# Autodesk Inventor assembly: Trunk
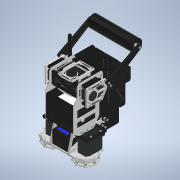
[picture p0: Inventor's stored thumbnail of the model, 180x180]
Saved by Autodesk Inventor 2020.4 (Build 244396000, 396)
## iProperties
Created: 2021-09-10
Part Number: Trunk
Document SubType Name: Assembly
Designer: Masato
Mass: 1705.67 g
Surface Area: 5977.9 cm^2
Volume: 961.439 cm^3
Density: 1.77408 g/cm^3
Author: Masato
## Documents named in this file (38)
- C:\Users\Masato\Documents\Inventor\CIT Brains_Inventor\OpenPlatform_ver3_0\UpperBody\Trunk\Trunk.iam
- C:\Users\Masato\Documents\Inventor\CIT Brains_Inventor\OpenPlatform_ver3_0\UpperBody\Trunk\Trunk_horizontal_frame_03.ipt
- C:\Users\Masato\Documents\Inventor\CIT Brains_Inventor\OpenPlatform_ver3_0\UpperBody\Trunk\Trunk_horizontal_frame_04.ipt
- C:\Users\Masato\Documents\Inventor\CIT Brains_Inventor\OpenPlatform_ver3_0\UpperBody\Trunk\Trunk_horizontal_frame_05.ipt
- C:\Users\Masato\Documents\Inventor\CIT Brains_Inventor\OpenPlatform_ver3_0\UpperBody\Trunk\Trunk_vertical_frame_02.ipt
- C:\Users\Masato\Documents\Inventor\CIT Brains_Inventor\OpenPlatform_ver3_0\UpperBody\Trunk\Trunk_vertical_frame_03.ipt
- C:\Users\Masato\Documents\Inventor\CIT Brains_Inventor\OpenPlatform_ver3_0\UpperBody\Trunk\Trunk_vertical_frame_04.ipt
- C:\Users\Masato\Documents\Inventor\CIT Brains_Inventor\OpenPlatform_ver3_0\UpperBody\Trunk\Trunk_vertical_frame_05.ipt
- C:\Users\Masato\Documents\Inventor\CIT Brains_Inventor\OpenPlatform_ver3_0\UpperBody\Trunk\Trunk_vertical_frame_06.ipt
- C:\Users\Masato\Documents\Inventor\CIT Brains_Inventor\OpenPlatform_ver3_0\Ready_Made\B3M11xx.ipt
- C:\Users\Masato\Documents\Inventor\CIT Brains_Inventor\OpenPlatform_ver3_0\Ready_Made\S3-07-3W.ipt
- C:\Users\Masato\Documents\Inventor\CIT Brains_Inventor\OpenPlatform_ver3_0\Ready_Made\ASU-375H.ipt
- C:\Users\Masato\Documents\Inventor\CIT Brains_Inventor\OpenPlatform_ver3_0\Ready_Made\B3M10xx.ipt
- C:\Users\Masato\Documents\Inventor\CIT Brains_Inventor\OpenPlatform_ver3_0\Ready_Made\SGB-100.ipt
- C:\Users\Masato\Documents\Inventor\CIT Brains_Inventor\OpenPlatform_ver3_0\UpperBody\Cockpit\Cockpit.iam
- C:\Users\Masato\Documents\Inventor\CIT Brains_Inventor\OpenPlatform_ver3_0\UpperBody\Trunk\Trunk_vertical_frame_04_MIR.ipt
- C:\Users\Masato\Documents\Inventor\CIT Brains_Inventor\OpenPlatform_ver3_0\UpperBody\Trunk\Trunk_vertical_frame_01.ipt
- C:\Users\Masato\Documents\Inventor\CIT Brains_Inventor\OpenPlatform_ver3_0\UpperBody\Trunk\Trunk_vertical_frame_01_MIR.ipt
- C:\Users\Masato\Documents\Inventor\CIT Brains_Inventor\OpenPlatform_ver3_0\Ready_Made\Screw\SPNFL-BRN-M3-6.ipt
- C:\Users\Masato\Documents\Inventor\CIT Brains_Inventor\OpenPlatform_ver3_0\Ready_Made\Screw\M2_6-15.ipt
- C:\Users\Masato\Documents\Inventor\CIT Brains_Inventor\OpenPlatform_ver3_0\Ready_Made\Screw\M3-8.ipt
- C:\Users\Masato\Documents\Inventor\CIT Brains_Inventor\OpenPlatform_ver3_0\Ready_Made\Screw\M3-6.ipt
- C:\Users\Masato\Documents\Inventor\CIT Brains_Inventor\OpenPlatform_ver3_0\Ready_Made\Screw\M2_6-20.ipt
- C:\Users\Masato\Documents\Inventor\CIT Brains_Inventor\OpenPlatform_ver3_0\UpperBody\Trunk\Outer_support_stand.ipt
- C:\Users\Masato\Documents\Inventor\CIT Brains_Inventor\OpenPlatform_ver3_0\Ready_Made\BRU-307S.ipt
- C:\Users\Masato\Documents\Inventor\CIT Brains_Inventor\OpenPlatform_ver3_0\UpperBody\Trunk\Outer_flange.ipt
- C:\Users\Masato\Documents\Inventor\CIT Brains_Inventor\OpenPlatform_ver3_0\UpperBody\Trunk\Inner_flange.ipt
- C:\Users\Masato\Documents\Inventor\CIT Brains_Inventor\OpenPlatform_ver3_0\Ready_Made\CRBA02508WWC8P5\CRBA02508WWC8P5.ipt
- C:\Users\Masato\Documents\Inventor\CIT Brains_Inventor\OpenPlatform_ver3_0\UpperBody\Trunk\Inner_support_stand.ipt
- C:\Users\Masato\Documents\Inventor\CIT Brains_Inventor\OpenPlatform_ver3_0\UpperBody\Trunk\Trunk_horizontal_frame_01.ipt
- C:\Users\Masato\Documents\Inventor\CIT Brains_Inventor\OpenPlatform_ver3_0\Ready_Made\SF319.ipt
- C:\Users\Masato\Documents\Inventor\CIT Brains_Inventor\OpenPlatform_ver3_0\Ready_Made\BRU-2609S.ipt
- C:\Users\Masato\Documents\Inventor\CIT Brains_Inventor\OpenPlatform_ver3_0\Ready_Made\Screw\M2_6-8.ipt
- C:\Users\Masato\Documents\Inventor\CIT Brains_Inventor\OpenPlatform_ver3_0\UpperBody\Trunk\Trunk_horizontal_frame_02.ipt
- C:\Users\Masato\Documents\Inventor\CIT Brains_Inventor\OpenPlatform_ver3_0\Ready_Made\UUW-0312-10BH.ipt
- C:\Users\Masato\Documents\Inventor\CIT Brains_Inventor\OpenPlatform_ver3_0\Ready_Made\Screw\M2_6-6.ipt
- C:\Users\Masato\Documents\Inventor\CIT Brains_Inventor\OpenPlatform_ver3_0\Ready_Made\ASU-309-6.ipt
- C:\Users\Masato\Documents\Inventor\CIT Brains_Inventor\OpenPlatform_ver3_0\Ready_Made\SLSBF7-131-M3-N3.ipt
## Components (229 placed, 37 different names)
1. Trunk_horizontal_frame_03:1 — 挿入:172, 挿入:173, 挿入:174, 挿入:175, 挿入:177, 挿入:179, 挿入:255, 挿入:256, 挿入:261, 挿入:262, 挿入:347, 挿入:348, 挿入:463, 挿入:464
2. Trunk_horizontal_frame_03:2 — 挿入:181, 挿入:182, 挿入:184, 挿入:185, 挿入:186, 挿入:187, 挿入:257, 挿入:258, 挿入:337, 挿入:338, 挿入:465, 挿入:466
3. Trunk_horizontal_frame_04:1 — 挿入:115, 挿入:116, 挿入:117, 挿入:118, 挿入:172, 挿入:173, 挿入:181, 挿入:182
4. Trunk_horizontal_frame_04:2 — 挿入:154, 挿入:155, 挿入:156, 挿入:157, 挿入:174, 挿入:175, 挿入:185, 挿入:187
5. Trunk_horizontal_frame_05:1 — 挿入:111, 挿入:112, 挿入:555, 挿入:556
6. Trunk_horizontal_frame_05:2 — 挿入:164, 挿入:165, 挿入:557, 挿入:558
7. Trunk_horizontal_frame_05:3 — 挿入:229, 挿入:230, 挿入:577, 挿入:579
8. Trunk_horizontal_frame_05:4 — 挿入:168, 挿入:169, 挿入:578, 挿入:580
9. Trunk_vertical_frame_01:1 — 角度:35, 角度:36, 挿入:200, 挿入:201, 挿入:420, 挿入:421, 挿入:426, 挿入:501, 挿入:502
10. Trunk_vertical_frame_01_MIR:1 — 角度:37, 角度:38, 挿入:202, 挿入:203, メイト:23, メイト:24, メイト:25, 挿入:418, 挿入:419, 挿入:499, 挿入:500
11. Trunk_vertical_frame_02:1 — フラッシュ:16, メイト:17, フラッシュ:18, フラッシュ:20, フラッシュ:21, メイト:22
12. Trunk_vertical_frame_02:2 — フラッシュ:16, メイト:17, フラッシュ:18, メイト:19
13. Trunk_vertical_frame_02:3 — フラッシュ:15, メイト:18, フラッシュ:17, フラッシュ:19, フラッシュ:20, フラッシュ:21, メイト:21, メイト:20
14. Trunk_vertical_frame_02:4 — フラッシュ:15, メイト:18, フラッシュ:17, メイト:25
15. Trunk_vertical_frame_03:1 — 挿入:101, 挿入:102, 挿入:103, 挿入:111, 挿入:112, 挿入:115, 挿入:116, 挿入:156, 挿入:157, 挿入:164, 挿入:165, フラッシュ:19, メイト:21, 挿入:208, 挿入:226, 挿入:245, 挿入:246, 挿入:247, 挿入:251, 挿入:252, 挿入:327, 挿入:328, 挿入:329, 挿入:330, 挿入:349, 挿入:350
16. Trunk_vertical_frame_03:2 — 挿入:104, 挿入:105, 挿入:106, 挿入:117, 挿入:118, 挿入:154, 挿入:155, 挿入:168, 挿入:169, メイト:22, 挿入:227, 挿入:229, 挿入:230, 挿入:248, 挿入:249, 挿入:250, 挿入:253, 挿入:254, 挿入:331, 挿入:332, 挿入:333, 挿入:334, 挿入:351, 挿入:352
17. Trunk_vertical_frame_04:1 — 挿入:555, 挿入:556, 挿入:557, 挿入:558, 挿入:559, 挿入:560, 挿入:561, 挿入:562, 挿入:563, 挿入:564, 挿入:565, 挿入:566, 挿入:567, 挿入:568, 挿入:569, 挿入:570, 角度:48, 挿入:571, 角度:49, 挿入:572, 挿入:573, 挿入:574
18. Trunk_vertical_frame_04_MIR:1 — 挿入:577, 挿入:578, 挿入:579, 挿入:580, 挿入:581, 挿入:582, 挿入:583, 挿入:584, 挿入:585, 挿入:586, 挿入:587, 挿入:588, 挿入:589, 挿入:590, 挿入:591, 挿入:592, 挿入:593, 挿入:594, 角度:50, 角度:51, 挿入:595, 挿入:596
19. Trunk_vertical_frame_05:1 — メイト:16, 挿入:263, 挿入:264, 挿入:267, 挿入:575, 挿入:576, 角度:52, 挿入:599
20. Trunk_vertical_frame_05:2 — 挿入:265, 挿入:266, 挿入:268, 挿入:597, 挿入:598
21. Trunk_vertical_frame_06:1 — 挿入:467, 挿入:468, 挿入:469, 挿入:470, 挿入:471, 挿入:472, 挿入:473, 挿入:474
22. Trunk_vertical_frame_06:2 — 挿入:475, 挿入:476, 挿入:477, 挿入:478, 挿入:479, 挿入:480, 挿入:481, 挿入:482
23. B3M11xx:1 — 角度:39, 挿入:391, 挿入:392, 挿入:422, 挿入:423, 挿入:424, 挿入:425, 挿入:483, 挿入:486
24. B3M11xx:2 — 挿入:427, 挿入:428, 挿入:429, 挿入:484, 挿入:485, 挿入:529
25. B3M11xx:3 — 挿入:177, 挿入:179, 挿入:184, 挿入:186
26. B3M10xx:4 — 挿入:475, 挿入:476, 挿入:477, 挿入:478, 挿入:559, 挿入:560, 挿入:561, 挿入:562
27. B3M10xx:5 — 挿入:467, 挿入:468, 挿入:469, 挿入:470, 挿入:581, 挿入:582, 挿入:583, 挿入:584
28. S3-07-3W:1 — 角度:37, 挿入:202
29. S3-07-3W:2 — 角度:38, 挿入:203
30. S3-07-3W:3 — 角度:36, 挿入:201
31. S3-07-3W:4 — 角度:35, 挿入:200
32. ASU-375H:1 — フラッシュ:9, フラッシュ:10, フラッシュ:11, フラッシュ:12, 挿入:101, 挿入:104, メイト:19, メイト:20, メイト:23, メイト:24
33. ASU-375H:2 — フラッシュ:9, フラッシュ:11, 挿入:102, 挿入:105
34. ASU-375H:3 — フラッシュ:10, フラッシュ:12, 挿入:103, 挿入:106
35. SGB-100:1 — メイト:16
36. Cockpit:1 [sub-assembly] — 挿入:208, 角度:39
37. SPNFL-BRN-M3-6:1 — 挿入:226
38. SPNFL-BRN-M3-6:2 — 挿入:227
39. M3-8:5 — 挿入:245
40. M3-8:6 — 挿入:246
41. M3-8:7 — 挿入:247
42. M3-8:8 — 挿入:248
43. M3-8:9 — 挿入:249
44. M3-8:10 — 挿入:250
45. M3-6:1 — 挿入:251
46. M3-6:2 — 挿入:252
47. M3-6:3 — 挿入:254
48. M3-6:4 — 挿入:253
49. M3-6:5 — 挿入:256
50. M3-6:6 — 挿入:255
51. M3-6:7 — 挿入:258
52. M3-6:8 — 挿入:257
53. M2_6-15:9 — 挿入:464
54. M2_6-15:10 — 挿入:463
55. M2_6-15:11 — 挿入:261
56. M2_6-15:12 — 挿入:262
57. M3-6:9 — 挿入:263
58. M3-6:10 — 挿入:264
59. M3-6:11 — 挿入:266
60. M3-6:12 — 挿入:265
61. M3-8:11 — 挿入:267
62. M3-8:12 — 挿入:268
63. M2_6-20:1 — 挿入:489
64. M2_6-20:2 — 挿入:490
65. M2_6-20:3 — 挿入:487
66. M2_6-20:4 — 挿入:488
67. M2_6-15:13 — 挿入:564
68. M2_6-15:14 — 挿入:563
69. M2_6-15:15 — 挿入:566
70. M2_6-15:16 — 挿入:565
71. M2_6-15:17 — 挿入:591
72. M2_6-15:18 — 挿入:592
73. M2_6-15:19 — 挿入:589
74. M2_6-15:20 — 挿入:590
75. M3-6:13 — 挿入:567
76. M3-6:14 — 挿入:568
77. M3-6:15 — 挿入:569
78. M3-6:16 — 挿入:570
79. M3-6:17 — 挿入:585
80. M3-6:18 — 挿入:586
81. M3-6:19 — 挿入:587
82. M3-6:20 — 挿入:588
83. M3-6:21 — 挿入:327
84. M3-6:22 — 挿入:328
85. M3-6:23 — 挿入:329
86. M3-6:24 — 挿入:330
87. M3-6:25 — 挿入:331
88. M3-6:26 — 挿入:332
89. M3-6:27 — 挿入:333
90. M3-6:28 — 挿入:334
91. M2_6-20:9 — 挿入:465
92. M2_6-20:10 — 挿入:466
93. M2_6-20:11 — 挿入:337
94. M2_6-20:12 — 挿入:338
95. M2_6-20:13 — 挿入:479
96. M2_6-20:14 — 挿入:482
97. M2_6-20:15 — 挿入:481
98. M2_6-20:16 — 挿入:480
99. M2_6-20:17 — 挿入:474
100. M2_6-20:18 — 挿入:472
101. M2_6-20:19 — 挿入:473
102. M2_6-20:20 — 挿入:471
103. M3-6:29 — 挿入:347
104. M3-6:30 — 挿入:348
105. M3-6:31 — 挿入:349
106. M3-6:32 — 挿入:350
107. M3-6:33 — 挿入:351
108. M3-6:34 — 挿入:352
109. Outer_support_stand:1 — 挿入:371, 挿入:372, 挿入:373, 挿入:374, 挿入:375, 挿入:376, 挿入:377, 挿入:378, 挿入:397, 挿入:438, 挿入:439
110. BRU-307S:1 — 挿入:371, 挿入:404
111. BRU-307S:2 — 挿入:372
112. BRU-307S:3 — 挿入:373
113. BRU-307S:4 — 挿入:374
114. BRU-307S:5 — 挿入:375, 挿入:405
115. BRU-307S:6 — 挿入:376
116. BRU-307S:7 — 挿入:377
117. BRU-307S:8 — 挿入:378
118. Inner_flange:1 — 挿入:391, 挿入:392, 挿入:452, 挿入:453, 挿入:454, 挿入:455
119. CRBA02508WWC8P5:1 — 挿入:397
120. Inner_support_stand:1 — 角度:40, 挿入:398, 角度:41, 挿入:399, 角度:42, 挿入:400, 角度:43, 挿入:401, 挿入:456, 挿入:457, 挿入:458, 挿入:459, 挿入:460, 挿入:461
121. S3-07-3W:9 — 角度:40, 挿入:398
122. S3-07-3W:10 — 角度:41, 挿入:399
123. S3-07-3W:11 — 角度:42, 挿入:400
124. S3-07-3W:12 — 角度:43, 挿入:401
125. Outer_flange:1 — 挿入:404, 挿入:405, 挿入:406, 挿入:407, 挿入:408, 挿入:409, 挿入:410, 挿入:411, 挿入:412, 挿入:413
126. M3-6:35 — 挿入:406
127. M3-6:36 — 挿入:407
128. M3-6:37 — 挿入:408
129. M3-6:38 — 挿入:409
130. M3-6:39 — 挿入:410
131. M3-6:40 — 挿入:411
132. M3-6:41 — 挿入:412
133. M3-6:42 — 挿入:413
134. Trunk_horizontal_frame_01:1 — 挿入:418, 挿入:419, 挿入:420, 挿入:421, 挿入:422, 挿入:423, 挿入:424, 挿入:425, 挿入:426, 挿入:427, 挿入:428, 挿入:429, 挿入:430, 挿入:431, 挿入:432, 挿入:433, 挿入:434, 挿入:435, 挿入:436, 挿入:440, 挿入:441, 挿入:442, 挿入:443, 挿入:444, 挿入:445, 挿入:446, 挿入:447, 挿入:448, 挿入:449, 挿入:450, 挿入:451, フラッシュ:22, 挿入:462, 挿入:511, 挿入:512, 挿入:513, 挿入:514, 挿入:515, 挿入:516, 挿入:517, 挿入:518
135. SF319:1 — 挿入:430
136. SF319:2 — 挿入:431
137. SF319:3 — 挿入:432
138. SF319:4 — 挿入:433, 挿入:439
139. SF319:5 — 挿入:434
140. SF319:6 — 挿入:435
141. SF319:7 — 挿入:436, 挿入:438
142. SF319:8 — 挿入:462
143. M2_6-15:21 — 挿入:441
144. M2_6-15:22 — 挿入:440
145. M2_6-15:23 — 挿入:442
146. M2_6-15:24 — 挿入:443
147. M2_6-15:25 — 挿入:444
148. M2_6-15:26 — 挿入:445
149. M2_6-15:27 — 挿入:446
150. M2_6-15:28 — 挿入:447
151. M3-8:13 — 挿入:448
152. M3-8:14 — 挿入:449
153. M3-8:15 — 挿入:450
154. M3-8:16 — 挿入:451
155. BRU-2609S:1 — 挿入:455, 挿入:457
156. BRU-2609S:2 — 挿入:454
157. BRU-2609S:3 — 挿入:453
158. BRU-2609S:4 — 挿入:452, 挿入:456
159. M2_6-8:1 — 挿入:458
160. M2_6-8:2 — 挿入:459
161. M2_6-8:3 — 挿入:460
162. M2_6-8:4 — 挿入:461
163. Trunk_horizontal_frame_02:1 — 挿入:483, 挿入:484, 挿入:485, 挿入:486, 挿入:487, 挿入:488, 挿入:489, 挿入:490
164. BRU-307S:9 — 挿入:497, 挿入:503
165. BRU-307S:10 — 挿入:498, 挿入:504
166. BRU-307S:11 — 挿入:496, 挿入:506
167. BRU-307S:12 — 挿入:495, 挿入:505
168. UUW-0312-10BH:1 — 挿入:495, 挿入:507
169. UUW-0312-10BH:2 — 挿入:496, 挿入:508
170. UUW-0312-10BH:3 — 挿入:497, 挿入:509
171. UUW-0312-10BH:4 — 挿入:498, 挿入:510
172. UUW-0312-10BH:5 — 挿入:499, 挿入:505
173. UUW-0312-10BH:6 — 挿入:500, 挿入:506
174. UUW-0312-10BH:7 — 挿入:501, 挿入:503
175. UUW-0312-10BH:8 — 挿入:502, 挿入:504
176. M3-6:43 — 挿入:507
177. M3-6:44 — 挿入:508
178. M3-6:45 — 挿入:510
179. M3-6:46 — 挿入:509
180. SF319:9 — 挿入:511, 挿入:519
181. SF319:10 — 挿入:512
182. SF319:11 — 挿入:513
183. SF319:12 — 挿入:514
184. SF319:13 — 挿入:515, 挿入:520
185. SF319:14 — 挿入:516
186. SF319:15 — 挿入:517
187. SF319:16 — 挿入:518
188. Outer_support_stand:2 — 挿入:519, 挿入:520, 挿入:521, 挿入:522, 挿入:523, 挿入:524, 挿入:525, 挿入:526, 挿入:527, 挿入:528, 挿入:554
189. BRU-307S:13 — 挿入:521, 挿入:534
190. BRU-307S:14 — 挿入:522
191. BRU-307S:15 — 挿入:523
192. BRU-307S:16 — 挿入:524
193. BRU-307S:17 — 挿入:525, 挿入:535
194. BRU-307S:18 — 挿入:526
195. BRU-307S:19 — 挿入:527
196. BRU-307S:20 — 挿入:528
197. BRU-2609S:5 — 挿入:530, 挿入:540
198. BRU-2609S:6 — 挿入:531, 挿入:541
199. BRU-2609S:7 — 挿入:532
200. BRU-2609S:8 — 挿入:533
201. S3-07-3W:13 — 角度:44, 挿入:536
202. S3-07-3W:14 — 角度:45, 挿入:537
203. S3-07-3W:15 — 角度:46, 挿入:538
204. S3-07-3W:16 — 角度:47, 挿入:539
205. Inner_flange:2 — 挿入:529, 挿入:530, 挿入:531, 挿入:532, 挿入:533
206. Inner_support_stand:2 — 角度:44, 挿入:536, 角度:45, 挿入:537, 角度:46, 挿入:538, 角度:47, 挿入:539, 挿入:540, 挿入:541, 挿入:550, 挿入:551, 挿入:552, 挿入:553
207. Outer_flange:2 — 挿入:534, 挿入:535, 挿入:542, 挿入:543, 挿入:544, 挿入:545, 挿入:546, 挿入:547, 挿入:548, 挿入:549
208. M3-6:47 — 挿入:542
209. M3-6:48 — 挿入:543
210. M3-6:49 — 挿入:544
211. M3-6:50 — 挿入:545
212. M3-6:51 — 挿入:546
213. M3-6:52 — 挿入:547
214. M3-6:53 — 挿入:548
215. M3-6:54 — 挿入:549
216. M2_6-6:1 — 挿入:550
217. M2_6-6:2 — 挿入:551
218. M2_6-6:3 — 挿入:552
219. M2_6-6:4 — 挿入:553
220. CRBA02508WWC8P5:2 — 挿入:554
221. ASU-309-6:1 — 角度:48, 挿入:571, 挿入:576
222. ASU-309-6:2 — 角度:49, 挿入:572, 挿入:575
223. M3-6:55 — 挿入:573
224. M3-6:56 — 挿入:574
225. M3-6:57 — 挿入:593
226. M3-6:58 — 挿入:594
227. ASU-309-6:3 — 角度:50, 挿入:595, 挿入:597
228. ASU-309-6:4 — 角度:51, 挿入:596, 挿入:598
229. SLSBF7-131-M3-N3:1 — 角度:52, 挿入:599
## Relationships (321: Insert 281, Angle 18, Flush 12, Mate 10)
- フラッシュ:9 [Flush]: ASU-375H:1 ↔ ASU-375H:2
- フラッシュ:10 [Flush]: ASU-375H:1 ↔ ASU-375H:3
- フラッシュ:11 [Flush]: ASU-375H:1 ↔ ASU-375H:2
- フラッシュ:12 [Flush]: ASU-375H:1 ↔ ASU-375H:3
- メイト:16 [Mate] (4 mm): Trunk_vertical_frame_05:1 ↔ SGB-100:1
- 挿入:101 [Insert]: Trunk_vertical_frame_03:1 ↔ ASU-375H:1
- 挿入:102 [Insert]: Trunk_vertical_frame_03:1 ↔ ASU-375H:2
- 挿入:103 [Insert]: Trunk_vertical_frame_03:1 ↔ ASU-375H:3
- 挿入:104 [Insert]: Trunk_vertical_frame_03:2 ↔ ASU-375H:1
- 挿入:105 [Insert]: Trunk_vertical_frame_03:2 ↔ ASU-375H:2
- 挿入:106 [Insert]: Trunk_vertical_frame_03:2 ↔ ASU-375H:3
- 挿入:111 [Insert]: Trunk_horizontal_frame_05:1 ↔ Trunk_vertical_frame_03:1
- 挿入:112 [Insert]: Trunk_horizontal_frame_05:1 ↔ Trunk_vertical_frame_03:1
- 挿入:115 [Insert]: Trunk_horizontal_frame_04:1 ↔ Trunk_vertical_frame_03:1
- 挿入:116 [Insert]: Trunk_horizontal_frame_04:1 ↔ Trunk_vertical_frame_03:1
- 挿入:117 [Insert]: Trunk_horizontal_frame_04:1 ↔ Trunk_vertical_frame_03:2
- 挿入:118 [Insert]: Trunk_horizontal_frame_04:1 ↔ Trunk_vertical_frame_03:2
- 挿入:154 [Insert]: Trunk_horizontal_frame_04:2 ↔ Trunk_vertical_frame_03:2
- 挿入:155 [Insert]: Trunk_horizontal_frame_04:2 ↔ Trunk_vertical_frame_03:2
- 挿入:156 [Insert]: Trunk_horizontal_frame_04:2 ↔ Trunk_vertical_frame_03:1
- 挿入:157 [Insert]: Trunk_horizontal_frame_04:2 ↔ Trunk_vertical_frame_03:1
- 挿入:164 [Insert]: Trunk_horizontal_frame_05:2 ↔ Trunk_vertical_frame_03:1
- 挿入:165 [Insert]: Trunk_horizontal_frame_05:2 ↔ Trunk_vertical_frame_03:1
- 挿入:168 [Insert]: Trunk_horizontal_frame_05:4 ↔ Trunk_vertical_frame_03:2
- 挿入:169 [Insert]: Trunk_horizontal_frame_05:4 ↔ Trunk_vertical_frame_03:2
- 挿入:172 [Insert]: Trunk_horizontal_frame_03:1 ↔ Trunk_horizontal_frame_04:1
- 挿入:173 [Insert]: Trunk_horizontal_frame_03:1 ↔ Trunk_horizontal_frame_04:1
- 挿入:174 [Insert]: Trunk_horizontal_frame_03:1 ↔ Trunk_horizontal_frame_04:2
- 挿入:175 [Insert]: Trunk_horizontal_frame_03:1 ↔ Trunk_horizontal_frame_04:2
- 挿入:177 [Insert]: Trunk_horizontal_frame_03:1 ↔ B3M11xx:3
- 挿入:179 [Insert]: Trunk_horizontal_frame_03:1 ↔ B3M11xx:3
- 挿入:181 [Insert]: Trunk_horizontal_frame_03:2 ↔ Trunk_horizontal_frame_04:1
- 挿入:182 [Insert]: Trunk_horizontal_frame_03:2 ↔ Trunk_horizontal_frame_04:1
- 挿入:184 [Insert]: Trunk_horizontal_frame_03:2 ↔ B3M11xx:3
- 挿入:185 [Insert]: Trunk_horizontal_frame_03:2 ↔ Trunk_horizontal_frame_04:2
- 挿入:186 [Insert]: Trunk_horizontal_frame_03:2 ↔ B3M11xx:3
- 挿入:187 [Insert]: Trunk_horizontal_frame_03:2 ↔ Trunk_horizontal_frame_04:2
- フラッシュ:15 [Flush]: Trunk_vertical_frame_02:3 ↔ Trunk_vertical_frame_02:4
- フラッシュ:16 [Flush]: Trunk_vertical_frame_02:1 ↔ Trunk_vertical_frame_02:2
- メイト:17 [Mate]: Trunk_vertical_frame_02:1 ↔ Trunk_vertical_frame_02:2
- メイト:18 [Mate]: Trunk_vertical_frame_02:3 ↔ Trunk_vertical_frame_02:4
- フラッシュ:17 [Flush]: Trunk_vertical_frame_02:3 ↔ Trunk_vertical_frame_02:4
- フラッシュ:18 [Flush]: Trunk_vertical_frame_02:1 ↔ Trunk_vertical_frame_02:2
- フラッシュ:19 [Flush]: Trunk_vertical_frame_02:3 ↔ Trunk_vertical_frame_03:1
- フラッシュ:20 [Flush]: Trunk_vertical_frame_02:1 ↔ Trunk_vertical_frame_02:3
- メイト:19 [Mate] (0.01 mm): Trunk_vertical_frame_02:2 ↔ ASU-375H:1
- メイト:20 [Mate] (0.01 mm): Trunk_vertical_frame_02:3 ↔ ASU-375H:1
- フラッシュ:21 [Flush]: Trunk_vertical_frame_02:1 ↔ Trunk_vertical_frame_02:3
- メイト:21 [Mate]: Trunk_vertical_frame_02:3 ↔ Trunk_vertical_frame_03:1
- メイト:22 [Mate]: Trunk_vertical_frame_02:1 ↔ Trunk_vertical_frame_03:2
- 角度:35 [Angle] (0 deg): Trunk_vertical_frame_01:1 ↔ S3-07-3W:4
- 角度:36 [Angle] (0 deg): Trunk_vertical_frame_01:1 ↔ S3-07-3W:3
- 挿入:200 [Insert]: Trunk_vertical_frame_01:1 ↔ S3-07-3W:4
- 挿入:201 [Insert]: Trunk_vertical_frame_01:1 ↔ S3-07-3W:3
- 角度:37 [Angle] (0 deg): Trunk_vertical_frame_01_MIR:1 ↔ S3-07-3W:1
- 角度:38 [Angle] (0 deg): Trunk_vertical_frame_01_MIR:1 ↔ S3-07-3W:2
- 挿入:202 [Insert]: Trunk_vertical_frame_01_MIR:1 ↔ S3-07-3W:1
- 挿入:203 [Insert]: Trunk_vertical_frame_01_MIR:1 ↔ S3-07-3W:2
- メイト:23 [Mate] (0.01 mm): Trunk_vertical_frame_01_MIR:1 ↔ ASU-375H:1
- メイト:24 [Mate] (0.01 mm): Trunk_vertical_frame_01_MIR:1 ↔ ASU-375H:1
- メイト:25 [Mate]: Trunk_vertical_frame_01_MIR:1 ↔ Trunk_vertical_frame_02:4
- 挿入:208 [Insert] (0.25 mm): Trunk_vertical_frame_03:1 ↔ Cockpit:1
- 角度:39 [Angle] (0 deg): B3M11xx:1 ↔ Cockpit:1
- 挿入:226 [Insert]: Trunk_vertical_frame_03:1 ↔ SPNFL-BRN-M3-6:1
- 挿入:227 [Insert]: Trunk_vertical_frame_03:2 ↔ SPNFL-BRN-M3-6:2
- 挿入:229 [Insert]: Trunk_horizontal_frame_05:3 ↔ Trunk_vertical_frame_03:2
- 挿入:230 [Insert]: Trunk_horizontal_frame_05:3 ↔ Trunk_vertical_frame_03:2
- 挿入:245 [Insert]: Trunk_vertical_frame_03:1 ↔ M3-8:5
- 挿入:246 [Insert]: Trunk_vertical_frame_03:1 ↔ M3-8:6
- 挿入:247 [Insert]: Trunk_vertical_frame_03:1 ↔ M3-8:7
- 挿入:248 [Insert]: Trunk_vertical_frame_03:2 ↔ M3-8:8
- 挿入:249 [Insert]: Trunk_vertical_frame_03:2 ↔ M3-8:9
- 挿入:250 [Insert]: Trunk_vertical_frame_03:2 ↔ M3-8:10
- 挿入:251 [Insert]: Trunk_vertical_frame_03:1 ↔ M3-6:1
- 挿入:252 [Insert]: Trunk_vertical_frame_03:1 ↔ M3-6:2
- 挿入:253 [Insert]: Trunk_vertical_frame_03:2 ↔ M3-6:4
- 挿入:254 [Insert]: Trunk_vertical_frame_03:2 ↔ M3-6:3
- 挿入:255 [Insert]: Trunk_horizontal_frame_03:1 ↔ M3-6:6
- 挿入:256 [Insert]: Trunk_horizontal_frame_03:1 ↔ M3-6:5
- 挿入:257 [Insert]: Trunk_horizontal_frame_03:2 ↔ M3-6:8
- 挿入:258 [Insert]: Trunk_horizontal_frame_03:2 ↔ M3-6:7
- 挿入:261 [Insert]: Trunk_horizontal_frame_03:1 ↔ M2_6-15:11
- 挿入:262 [Insert]: Trunk_horizontal_frame_03:1 ↔ M2_6-15:12
- 挿入:263 [Insert]: Trunk_vertical_frame_05:1 ↔ M3-6:9
- 挿入:264 [Insert]: Trunk_vertical_frame_05:1 ↔ M3-6:10
- 挿入:265 [Insert]: Trunk_vertical_frame_05:2 ↔ M3-6:12
- 挿入:266 [Insert]: Trunk_vertical_frame_05:2 ↔ M3-6:11
- 挿入:267 [Insert]: Trunk_vertical_frame_05:1 ↔ M3-8:11
- 挿入:268 [Insert]: Trunk_vertical_frame_05:2 ↔ M3-8:12
- 挿入:327 [Insert]: Trunk_vertical_frame_03:1 ↔ M3-6:21
- 挿入:328 [Insert]: Trunk_vertical_frame_03:1 ↔ M3-6:22
- 挿入:329 [Insert]: Trunk_vertical_frame_03:1 ↔ M3-6:23
- 挿入:330 [Insert]: Trunk_vertical_frame_03:1 ↔ M3-6:24
- 挿入:331 [Insert]: Trunk_vertical_frame_03:2 ↔ M3-6:25
- 挿入:332 [Insert]: Trunk_vertical_frame_03:2 ↔ M3-6:26
- 挿入:333 [Insert]: Trunk_vertical_frame_03:2 ↔ M3-6:27
- 挿入:334 [Insert]: Trunk_vertical_frame_03:2 ↔ M3-6:28
- 挿入:337 [Insert]: Trunk_horizontal_frame_03:2 ↔ M2_6-20:11
- 挿入:338 [Insert]: Trunk_horizontal_frame_03:2 ↔ M2_6-20:12
- 挿入:347 [Insert]: Trunk_horizontal_frame_03:1 ↔ M3-6:29
- 挿入:348 [Insert]: Trunk_horizontal_frame_03:1 ↔ M3-6:30
- 挿入:349 [Insert]: Trunk_vertical_frame_03:1 ↔ M3-6:31
- 挿入:350 [Insert]: Trunk_vertical_frame_03:1 ↔ M3-6:32
- 挿入:351 [Insert]: Trunk_vertical_frame_03:2 ↔ M3-6:33
- 挿入:352 [Insert]: Trunk_vertical_frame_03:2 ↔ M3-6:34
- 挿入:371 [Insert]: Outer_support_stand:1 ↔ BRU-307S:1
- 挿入:372 [Insert]: Outer_support_stand:1 ↔ BRU-307S:2
- 挿入:373 [Insert]: Outer_support_stand:1 ↔ BRU-307S:3
- 挿入:374 [Insert]: Outer_support_stand:1 ↔ BRU-307S:4
- 挿入:375 [Insert]: Outer_support_stand:1 ↔ BRU-307S:5
- 挿入:376 [Insert]: Outer_support_stand:1 ↔ BRU-307S:6
- 挿入:377 [Insert]: Outer_support_stand:1 ↔ BRU-307S:7
- 挿入:378 [Insert]: Outer_support_stand:1 ↔ BRU-307S:8
- 挿入:391 [Insert]: B3M11xx:1 ↔ Inner_flange:1
- 挿入:392 [Insert]: B3M11xx:1 ↔ Inner_flange:1
- 挿入:397 [Insert]: Outer_support_stand:1 ↔ CRBA02508WWC8P5:1
- 角度:40 [Angle] (0 deg): Inner_support_stand:1 ↔ S3-07-3W:9
- 挿入:398 [Insert]: Inner_support_stand:1 ↔ S3-07-3W:9
- 角度:41 [Angle] (0 deg): Inner_support_stand:1 ↔ S3-07-3W:10
- 挿入:399 [Insert]: Inner_support_stand:1 ↔ S3-07-3W:10
- 角度:42 [Angle] (0 deg): Inner_support_stand:1 ↔ S3-07-3W:11
- 挿入:400 [Insert]: Inner_support_stand:1 ↔ S3-07-3W:11
- 角度:43 [Angle] (0 deg): Inner_support_stand:1 ↔ S3-07-3W:12
- 挿入:401 [Insert]: Inner_support_stand:1 ↔ S3-07-3W:12
- 挿入:404 [Insert]: BRU-307S:1 ↔ Outer_flange:1
- 挿入:405 [Insert]: BRU-307S:5 ↔ Outer_flange:1
- 挿入:406 [Insert]: Outer_flange:1 ↔ M3-6:35
- 挿入:407 [Insert]: Outer_flange:1 ↔ M3-6:36
- 挿入:408 [Insert]: Outer_flange:1 ↔ M3-6:37
- 挿入:409 [Insert]: Outer_flange:1 ↔ M3-6:38
- 挿入:410 [Insert]: Outer_flange:1 ↔ M3-6:39
- 挿入:411 [Insert]: Outer_flange:1 ↔ M3-6:40
- 挿入:412 [Insert]: Outer_flange:1 ↔ M3-6:41
- 挿入:413 [Insert]: Outer_flange:1 ↔ M3-6:42
- 挿入:418 [Insert]: Trunk_vertical_frame_01_MIR:1 ↔ Trunk_horizontal_frame_01:1
- 挿入:419 [Insert]: Trunk_vertical_frame_01_MIR:1 ↔ Trunk_horizontal_frame_01:1
- 挿入:420 [Insert]: Trunk_vertical_frame_01:1 ↔ Trunk_horizontal_frame_01:1
- 挿入:421 [Insert]: Trunk_vertical_frame_01:1 ↔ Trunk_horizontal_frame_01:1
- 挿入:422 [Insert]: B3M11xx:1 ↔ Trunk_horizontal_frame_01:1
- 挿入:423 [Insert]: B3M11xx:1 ↔ Trunk_horizontal_frame_01:1
- 挿入:424 [Insert]: B3M11xx:1 ↔ Trunk_horizontal_frame_01:1
- 挿入:425 [Insert]: B3M11xx:1 ↔ Trunk_horizontal_frame_01:1
- 挿入:426 [Insert]: Trunk_vertical_frame_01:1 ↔ Trunk_horizontal_frame_01:1
- 挿入:427 [Insert]: B3M11xx:2 ↔ Trunk_horizontal_frame_01:1
- 挿入:428 [Insert]: B3M11xx:2 ↔ Trunk_horizontal_frame_01:1
- 挿入:429 [Insert]: B3M11xx:2 ↔ Trunk_horizontal_frame_01:1
- 挿入:430 [Insert]: Trunk_horizontal_frame_01:1 ↔ SF319:1
- 挿入:431 [Insert]: Trunk_horizontal_frame_01:1 ↔ SF319:2
- 挿入:432 [Insert]: Trunk_horizontal_frame_01:1 ↔ SF319:3
- 挿入:433 [Insert]: Trunk_horizontal_frame_01:1 ↔ SF319:4
- 挿入:434 [Insert]: Trunk_horizontal_frame_01:1 ↔ SF319:5
- 挿入:435 [Insert]: Trunk_horizontal_frame_01:1 ↔ SF319:6
- 挿入:436 [Insert]: Trunk_horizontal_frame_01:1 ↔ SF319:7
- 挿入:438 [Insert]: Outer_support_stand:1 ↔ SF319:7
- 挿入:439 [Insert]: Outer_support_stand:1 ↔ SF319:4
- 挿入:440 [Insert]: Trunk_horizontal_frame_01:1 ↔ M2_6-15:22
- 挿入:441 [Insert]: Trunk_horizontal_frame_01:1 ↔ M2_6-15:21
- 挿入:442 [Insert]: Trunk_horizontal_frame_01:1 ↔ M2_6-15:23
- 挿入:443 [Insert]: Trunk_horizontal_frame_01:1 ↔ M2_6-15:24
- 挿入:444 [Insert]: Trunk_horizontal_frame_01:1 ↔ M2_6-15:25
- 挿入:445 [Insert]: Trunk_horizontal_frame_01:1 ↔ M2_6-15:26
- 挿入:446 [Insert]: Trunk_horizontal_frame_01:1 ↔ M2_6-15:27
- 挿入:447 [Insert]: Trunk_horizontal_frame_01:1 ↔ M2_6-15:28
- 挿入:448 [Insert]: Trunk_horizontal_frame_01:1 ↔ M3-8:13
- 挿入:449 [Insert]: Trunk_horizontal_frame_01:1 ↔ M3-8:14
- 挿入:450 [Insert]: Trunk_horizontal_frame_01:1 ↔ M3-8:15
- 挿入:451 [Insert]: Trunk_horizontal_frame_01:1 ↔ M3-8:16
- 挿入:452 [Insert]: Inner_flange:1 ↔ BRU-2609S:4
- 挿入:453 [Insert]: Inner_flange:1 ↔ BRU-2609S:3
- 挿入:454 [Insert]: Inner_flange:1 ↔ BRU-2609S:2
- 挿入:455 [Insert]: Inner_flange:1 ↔ BRU-2609S:1
- 挿入:456 [Insert]: Inner_support_stand:1 ↔ BRU-2609S:4
- 挿入:457 [Insert]: Inner_support_stand:1 ↔ BRU-2609S:1
- 挿入:458 [Insert]: Inner_support_stand:1 ↔ M2_6-8:1
- 挿入:459 [Insert]: Inner_support_stand:1 ↔ M2_6-8:2
- 挿入:460 [Insert]: Inner_support_stand:1 ↔ M2_6-8:3
- 挿入:461 [Insert]: Inner_support_stand:1 ↔ M2_6-8:4
- フラッシュ:22 [Flush]: Trunk_horizontal_frame_01:1
- 挿入:462 [Insert]: Trunk_horizontal_frame_01:1 ↔ SF319:8
- 挿入:463 [Insert]: Trunk_horizontal_frame_03:1 ↔ M2_6-15:10
- 挿入:464 [Insert]: Trunk_horizontal_frame_03:1 ↔ M2_6-15:9
- 挿入:465 [Insert]: Trunk_horizontal_frame_03:2 ↔ M2_6-20:9
- 挿入:466 [Insert]: Trunk_horizontal_frame_03:2 ↔ M2_6-20:10
- 挿入:467 [Insert]: Trunk_vertical_frame_06:1 ↔ B3M10xx:5
- 挿入:468 [Insert]: Trunk_vertical_frame_06:1 ↔ B3M10xx:5
- 挿入:469 [Insert]: Trunk_vertical_frame_06:1 ↔ B3M10xx:5
- 挿入:470 [Insert]: Trunk_vertical_frame_06:1 ↔ B3M10xx:5
- 挿入:471 [Insert]: Trunk_vertical_frame_06:1 ↔ M2_6-20:20
- 挿入:472 [Insert]: Trunk_vertical_frame_06:1 ↔ M2_6-20:18
- 挿入:473 [Insert]: Trunk_vertical_frame_06:1 ↔ M2_6-20:19
- 挿入:474 [Insert]: Trunk_vertical_frame_06:1 ↔ M2_6-20:17
- 挿入:475 [Insert]: Trunk_vertical_frame_06:2 ↔ B3M10xx:4
- 挿入:476 [Insert]: Trunk_vertical_frame_06:2 ↔ B3M10xx:4
- 挿入:477 [Insert]: Trunk_vertical_frame_06:2 ↔ B3M10xx:4
- 挿入:478 [Insert]: Trunk_vertical_frame_06:2 ↔ B3M10xx:4
- 挿入:479 [Insert]: Trunk_vertical_frame_06:2 ↔ M2_6-20:13
- 挿入:480 [Insert]: Trunk_vertical_frame_06:2 ↔ M2_6-20:16
- 挿入:481 [Insert]: Trunk_vertical_frame_06:2 ↔ M2_6-20:15
- 挿入:482 [Insert]: Trunk_vertical_frame_06:2 ↔ M2_6-20:14
- 挿入:483 [Insert]: B3M11xx:1 ↔ Trunk_horizontal_frame_02:1
- 挿入:484 [Insert]: B3M11xx:2 ↔ Trunk_horizontal_frame_02:1
- 挿入:485 [Insert]: B3M11xx:2 ↔ Trunk_horizontal_frame_02:1
- 挿入:486 [Insert]: B3M11xx:1 ↔ Trunk_horizontal_frame_02:1
- 挿入:487 [Insert]: M2_6-20:3 ↔ Trunk_horizontal_frame_02:1
- 挿入:488 [Insert]: M2_6-20:4 ↔ Trunk_horizontal_frame_02:1
- 挿入:489 [Insert]: M2_6-20:1 ↔ Trunk_horizontal_frame_02:1
- 挿入:490 [Insert]: M2_6-20:2 ↔ Trunk_horizontal_frame_02:1
- 挿入:495 [Insert]: BRU-307S:12 ↔ UUW-0312-10BH:1
- 挿入:496 [Insert]: BRU-307S:11 ↔ UUW-0312-10BH:2
- 挿入:497 [Insert]: BRU-307S:9 ↔ UUW-0312-10BH:3
- 挿入:498 [Insert]: BRU-307S:10 ↔ UUW-0312-10BH:4
- 挿入:499 [Insert]: Trunk_vertical_frame_01_MIR:1 ↔ UUW-0312-10BH:5
- 挿入:500 [Insert]: Trunk_vertical_frame_01_MIR:1 ↔ UUW-0312-10BH:6
- 挿入:501 [Insert]: Trunk_vertical_frame_01:1 ↔ UUW-0312-10BH:7
- 挿入:502 [Insert]: Trunk_vertical_frame_01:1 ↔ UUW-0312-10BH:8
- 挿入:503 [Insert]: BRU-307S:9 ↔ UUW-0312-10BH:7
- 挿入:504 [Insert]: BRU-307S:10 ↔ UUW-0312-10BH:8
- 挿入:505 [Insert]: BRU-307S:12 ↔ UUW-0312-10BH:5
- 挿入:506 [Insert]: BRU-307S:11 ↔ UUW-0312-10BH:6
- 挿入:507 [Insert]: UUW-0312-10BH:1 ↔ M3-6:43
- 挿入:508 [Insert]: UUW-0312-10BH:2 ↔ M3-6:44
- 挿入:509 [Insert]: UUW-0312-10BH:3 ↔ M3-6:46
- 挿入:510 [Insert]: UUW-0312-10BH:4 ↔ M3-6:45
- 挿入:511 [Insert]: Trunk_horizontal_frame_01:1 ↔ SF319:9
- 挿入:512 [Insert]: Trunk_horizontal_frame_01:1 ↔ SF319:10
- 挿入:513 [Insert]: Trunk_horizontal_frame_01:1 ↔ SF319:11
- 挿入:514 [Insert]: Trunk_horizontal_frame_01:1 ↔ SF319:12
- 挿入:515 [Insert]: Trunk_horizontal_frame_01:1 ↔ SF319:13
- 挿入:516 [Insert]: Trunk_horizontal_frame_01:1 ↔ SF319:14
- 挿入:517 [Insert]: Trunk_horizontal_frame_01:1 ↔ SF319:15
- 挿入:518 [Insert]: Trunk_horizontal_frame_01:1 ↔ SF319:16
- 挿入:519 [Insert]: SF319:9 ↔ Outer_support_stand:2
- 挿入:520 [Insert]: SF319:13 ↔ Outer_support_stand:2
- 挿入:521 [Insert]: Outer_support_stand:2 ↔ BRU-307S:13
- 挿入:522 [Insert]: Outer_support_stand:2 ↔ BRU-307S:14
- 挿入:523 [Insert]: Outer_support_stand:2 ↔ BRU-307S:15
- 挿入:524 [Insert]: Outer_support_stand:2 ↔ BRU-307S:16
- 挿入:525 [Insert]: Outer_support_stand:2 ↔ BRU-307S:17
- 挿入:526 [Insert]: Outer_support_stand:2 ↔ BRU-307S:18
- 挿入:527 [Insert]: Outer_support_stand:2 ↔ BRU-307S:19
- 挿入:528 [Insert]: Outer_support_stand:2 ↔ BRU-307S:20
- 挿入:529 [Insert]: B3M11xx:2 ↔ Inner_flange:2
- 挿入:530 [Insert]: BRU-2609S:5 ↔ Inner_flange:2
- 挿入:531 [Insert]: BRU-2609S:6 ↔ Inner_flange:2
- 挿入:532 [Insert]: BRU-2609S:7 ↔ Inner_flange:2
- 挿入:533 [Insert]: BRU-2609S:8 ↔ Inner_flange:2
- 挿入:534 [Insert]: BRU-307S:13 ↔ Outer_flange:2
- 挿入:535 [Insert]: BRU-307S:17 ↔ Outer_flange:2
- 角度:44 [Angle] (0 deg): S3-07-3W:13 ↔ Inner_support_stand:2
- 挿入:536 [Insert]: S3-07-3W:13 ↔ Inner_support_stand:2
- 角度:45 [Angle] (0 deg): S3-07-3W:14 ↔ Inner_support_stand:2
- 挿入:537 [Insert]: S3-07-3W:14 ↔ Inner_support_stand:2
- 角度:46 [Angle] (0 deg): S3-07-3W:15 ↔ Inner_support_stand:2
- 挿入:538 [Insert]: S3-07-3W:15 ↔ Inner_support_stand:2
- 角度:47 [Angle] (0 deg): S3-07-3W:16 ↔ Inner_support_stand:2
- 挿入:539 [Insert]: S3-07-3W:16 ↔ Inner_support_stand:2
- 挿入:540 [Insert]: BRU-2609S:5 ↔ Inner_support_stand:2
- 挿入:541 [Insert]: BRU-2609S:6 ↔ Inner_support_stand:2
- 挿入:542 [Insert]: Outer_flange:2 ↔ M3-6:47
- 挿入:543 [Insert]: Outer_flange:2 ↔ M3-6:48
- 挿入:544 [Insert]: Outer_flange:2 ↔ M3-6:49
- 挿入:545 [Insert]: Outer_flange:2 ↔ M3-6:50
- 挿入:546 [Insert]: Outer_flange:2 ↔ M3-6:51
- 挿入:547 [Insert]: Outer_flange:2 ↔ M3-6:52
- 挿入:548 [Insert]: Outer_flange:2 ↔ M3-6:53
- 挿入:549 [Insert]: Outer_flange:2 ↔ M3-6:54
- 挿入:550 [Insert]: Inner_support_stand:2 ↔ M2_6-6:1
- 挿入:551 [Insert]: Inner_support_stand:2 ↔ M2_6-6:2
- 挿入:552 [Insert]: Inner_support_stand:2 ↔ M2_6-6:3
- 挿入:553 [Insert]: Inner_support_stand:2 ↔ M2_6-6:4
- 挿入:554 [Insert]: Outer_support_stand:2 ↔ CRBA02508WWC8P5:2
- 挿入:555 [Insert]: Trunk_horizontal_frame_05:1 ↔ Trunk_vertical_frame_04:1
- 挿入:556 [Insert]: Trunk_horizontal_frame_05:1 ↔ Trunk_vertical_frame_04:1
- 挿入:557 [Insert]: Trunk_horizontal_frame_05:2 ↔ Trunk_vertical_frame_04:1
- 挿入:558 [Insert]: Trunk_horizontal_frame_05:2 ↔ Trunk_vertical_frame_04:1
- 挿入:559 [Insert]: Trunk_vertical_frame_04:1 ↔ B3M10xx:4
- 挿入:560 [Insert]: Trunk_vertical_frame_04:1 ↔ B3M10xx:4
- 挿入:561 [Insert]: Trunk_vertical_frame_04:1 ↔ B3M10xx:4
- 挿入:562 [Insert]: Trunk_vertical_frame_04:1 ↔ B3M10xx:4
- 挿入:563 [Insert]: Trunk_vertical_frame_04:1 ↔ M2_6-15:14
- 挿入:564 [Insert]: Trunk_vertical_frame_04:1 ↔ M2_6-15:13
- 挿入:565 [Insert]: Trunk_vertical_frame_04:1 ↔ M2_6-15:16
- 挿入:566 [Insert]: Trunk_vertical_frame_04:1 ↔ M2_6-15:15
- 挿入:567 [Insert]: Trunk_vertical_frame_04:1 ↔ M3-6:13
- 挿入:568 [Insert]: Trunk_vertical_frame_04:1 ↔ M3-6:14
- 挿入:569 [Insert]: Trunk_vertical_frame_04:1 ↔ M3-6:15
- 挿入:570 [Insert]: Trunk_vertical_frame_04:1 ↔ M3-6:16
- 角度:48 [Angle] (0 deg): Trunk_vertical_frame_04:1 ↔ ASU-309-6:1
- 挿入:571 [Insert]: Trunk_vertical_frame_04:1 ↔ ASU-309-6:1
- 角度:49 [Angle] (0 deg): Trunk_vertical_frame_04:1 ↔ ASU-309-6:2
- 挿入:572 [Insert]: Trunk_vertical_frame_04:1 ↔ ASU-309-6:2
- 挿入:573 [Insert]: Trunk_vertical_frame_04:1 ↔ M3-6:55
- 挿入:574 [Insert]: Trunk_vertical_frame_04:1 ↔ M3-6:56
- 挿入:575 [Insert]: Trunk_vertical_frame_05:1 ↔ ASU-309-6:2
- 挿入:576 [Insert]: Trunk_vertical_frame_05:1 ↔ ASU-309-6:1
- 挿入:577 [Insert]: Trunk_horizontal_frame_05:3 ↔ Trunk_vertical_frame_04_MIR:1
- 挿入:578 [Insert]: Trunk_horizontal_frame_05:4 ↔ Trunk_vertical_frame_04_MIR:1
- 挿入:579 [Insert]: Trunk_horizontal_frame_05:3 ↔ Trunk_vertical_frame_04_MIR:1
- 挿入:580 [Insert]: Trunk_horizontal_frame_05:4 ↔ Trunk_vertical_frame_04_MIR:1
- 挿入:581 [Insert]: Trunk_vertical_frame_04_MIR:1 ↔ B3M10xx:5
- 挿入:582 [Insert]: Trunk_vertical_frame_04_MIR:1 ↔ B3M10xx:5
- 挿入:583 [Insert]: Trunk_vertical_frame_04_MIR:1 ↔ B3M10xx:5
- 挿入:584 [Insert]: Trunk_vertical_frame_04_MIR:1 ↔ B3M10xx:5
- 挿入:585 [Insert]: Trunk_vertical_frame_04_MIR:1 ↔ M3-6:17
- 挿入:586 [Insert]: Trunk_vertical_frame_04_MIR:1 ↔ M3-6:18
- 挿入:587 [Insert]: Trunk_vertical_frame_04_MIR:1 ↔ M3-6:19
- 挿入:588 [Insert]: Trunk_vertical_frame_04_MIR:1 ↔ M3-6:20
- 挿入:589 [Insert]: Trunk_vertical_frame_04_MIR:1 ↔ M2_6-15:19
- 挿入:590 [Insert]: Trunk_vertical_frame_04_MIR:1 ↔ M2_6-15:20
- 挿入:591 [Insert]: Trunk_vertical_frame_04_MIR:1 ↔ M2_6-15:17
- 挿入:592 [Insert]: Trunk_vertical_frame_04_MIR:1 ↔ M2_6-15:18
- 挿入:593 [Insert]: Trunk_vertical_frame_04_MIR:1 ↔ M3-6:57
- 挿入:594 [Insert]: Trunk_vertical_frame_04_MIR:1 ↔ M3-6:58
- 角度:50 [Angle] (0 deg): Trunk_vertical_frame_04_MIR:1 ↔ ASU-309-6:3
- 角度:51 [Angle] (0 deg): Trunk_vertical_frame_04_MIR:1 ↔ ASU-309-6:4
- 挿入:595 [Insert]: Trunk_vertical_frame_04_MIR:1 ↔ ASU-309-6:3
- 挿入:596 [Insert]: Trunk_vertical_frame_04_MIR:1 ↔ ASU-309-6:4
- 挿入:597 [Insert]: Trunk_vertical_frame_05:2 ↔ ASU-309-6:3
- 挿入:598 [Insert]: Trunk_vertical_frame_05:2 ↔ ASU-309-6:4
- 角度:52 [Angle] (0 deg): Trunk_vertical_frame_05:1 ↔ SLSBF7-131-M3-N3:1
- 挿入:599 [Insert]: Trunk_vertical_frame_05:1 ↔ SLSBF7-131-M3-N3:1
